# Autodesk Inventor assembly: Chasis
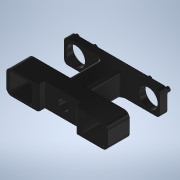
[picture p0: Inventor's stored thumbnail of the model, 180x180]
Saved by Autodesk Inventor 2022 (Build 260153000, 153)
## iProperties
Created: 2021-11-24
Part Number: Chasis
Document SubType Name: Assembly
Designer: JK
Author: JK
## Documents named in this file (3)
- C:\Users\JK\Documents\Inventor\N20 Leg Actuator\N20-Leg-Actuator\CADfiles\Chasis.iam
- C:\Users\JK\Documents\Inventor\N20 Leg Actuator\N20-Leg-Actuator\CADfiles\Base.ipt
- C:\Users\JK\Documents\Inventor\N20 Leg Actuator\N20-Leg-Actuator\CADfiles\PotHolder.ipt
## Components (2 placed, 2 different names)
1. Base:1 — Nivelación:1, Coincidencia:2
2. PotHolder:1 — Nivelación:1, Coincidencia:2
## Relationships (4: Mate 2, Angle 1, Flush 1)
- [Angle] (0 deg): Base:1 ↔ PotHolder:1
- [Mate]: Base:1 ↔ PotHolder:1
- Nivelación:1 [Flush]: Base:1 ↔ PotHolder:1
- Coincidencia:2 [Mate]: Base:1 ↔ PotHolder:1
